# Autodesk Inventor assembly: Assembly w draft-end
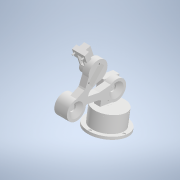
[picture p0: Inventor's stored thumbnail of the model, 180x180]
Saved by Autodesk Inventor 2022 (Build 260153000, 153)
## iProperties
Created: 2022-02-11
Part Number: Assembly w draft-end
Document SubType Name: Assembly
Designer: Alexa
Author: Alexa
## Documents named in this file (6)
- C:\Users\Alexa\Documents\4TH YEAR\ROBOTICS PARTS\NEW PARTS\Assembly w draft-end.iam
- C:\Users\Alexa\Documents\4TH YEAR\ROBOTICS PARTS\NEW PARTS\NBase Part.ipt
- C:\Users\Alexa\Documents\4TH YEAR\ROBOTICS PARTS\NEW PARTS\NBase top.ipt
- C:\Users\Alexa\Documents\4TH YEAR\ROBOTICS PARTS\NEW PARTS\1stArm.ipt
- C:\Users\Alexa\Documents\4TH YEAR\ROBOTICS PARTS\NEW PARTS\2ndArm.ipt
- C:\Users\Alexa\Documents\4TH YEAR\ROBOTICS PARTS\NEW PARTS\EndConnector.ipt
## Components (5 placed, 5 different names)
1. NBase Part:1 — Rotational:1
2. NBase top:1 — Rotational:1, Rotational:2
3. 1stArm:1 — Rotational:2, Rotational:3
4. 2ndArm:1 — Rotational:3, Rotational:4
5. EndConnector:1 — Rotational:4
## Relationships (4: RevoluteJoint 4)
- Rotational:1 [RevoluteJoint]: NBase Part:1 ↔ NBase top:1
- Rotational:2 [RevoluteJoint]: NBase top:1 ↔ 1stArm:1
- Rotational:3 [RevoluteJoint]: 1stArm:1 ↔ 2ndArm:1
- Rotational:4 [RevoluteJoint]: 2ndArm:1 ↔ EndConnector:1
